# Autodesk Inventor assembly: Assembly8 (Cylinder Complete Sub Assembly)
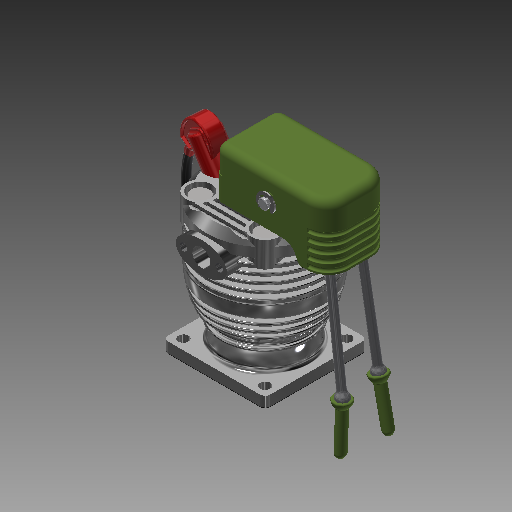
[picture p0: Inventor's stored thumbnail of the model, 512x512]
Saved by Autodesk Inventor 2018 (Build 220112000, 112)
## iProperties
Created: 2023-05-02
Part Number: Assembly8 (Cylinder Complete Sub Assembly)
Document SubType Name: Assembly
Designer: Habib Mohamed
Author: Habib Mohamed
## Documents named in this file (10)
- D:\Inventor\My projects\Rotary Engine\Assembly\Assembly8 (Cylinder Complete Sub Assembly).iam
- D:\Inventor\My projects\Rotary Engine\Component 48(Ignition Plug).ipt
- D:\Inventor\My projects\Rotary Engine\Component 45(Spark Plug).ipt
- D:\Inventor\My projects\Rotary Engine\Component 4 (Pound).ipt
- D:\Inventor\My projects\Rotary Engine\Component 39(Rod).ipt
- D:\Inventor\My projects\Rotary Engine\Assembly\Assembly7.iam
- Cykinder SubAssembly.iam
- D:\Inventor\My projects\Rotary Engine\Assembly\Assembly3(Rocker arm Sub Assembly).iam
- D:\Inventor\My projects\Rotary Engine\Assembly\Assembly5 (Valve Sub Assembly).iam
- D:\Inventor\My projects\Rotary Engine\Component 27 (Bracket Cover).ipt
## Components (12 placed, 8 different names)
1. Component 48(Ignition Plug):1 — Mate:1, Mate:2, Mate:3
2. Component 45(Spark Plug):1 — Mate:1, Mate:2, Mate:3, Mate:4, Mate:5
3. Component 4 (Pound):1 — Tangent:2
4. Component 39(Rod):1 — Tangent:2, Tangent:4
5. Component 4 (Pound):2 — Tangent:1
6. Component 39(Rod):2 — Tangent:1, Tangent:3
7. Cykinder SubAssembly:1 [sub-assembly] — Mate:4, Mate:5, Mate:6, Mate:7, Mate:8, Mate:9, Mate:10, Mate:11, Mate:12, Mate:13, Mate:14, Mate:15, Flush:1
8. Assembly3(Rocker arm Sub Assembly):1 [sub-assembly] — Mate:11, Mate:12, Tangent:4
9. Assembly5 (Valve Sub Assembly):1 [sub-assembly] — Mate:6, Mate:8
10. Assembly3(Rocker arm Sub Assembly):2 [sub-assembly] — Mate:10, Mate:13, Tangent:3
11. Assembly5 (Valve Sub Assembly):2 [sub-assembly] — Mate:7, Mate:9
12. Component 27 (Bracket Cover):1 — Mate:14, Mate:15, Flush:1
## Relationships (20: Mate 15, Tangent 4, Flush 1)
- Mate:1: Component 48(Ignition Plug):1 ↔ Component 45(Spark Plug):1
- Mate:2: Component 48(Ignition Plug):1 ↔ Component 45(Spark Plug):1
- Mate:3: Component 48(Ignition Plug):1 ↔ Component 45(Spark Plug):1
- Mate:4: Component 45(Spark Plug):1 ↔ Cykinder SubAssembly:1
- Mate:5: Component 45(Spark Plug):1 ↔ Cykinder SubAssembly:1
- Mate:6: Cykinder SubAssembly:1 ↔ Assembly5 (Valve Sub Assembly):1
- Mate:7: Cykinder SubAssembly:1 ↔ Assembly5 (Valve Sub Assembly):2
- Mate:8: Cykinder SubAssembly:1 ↔ Assembly5 (Valve Sub Assembly):1
- Mate:9: Cykinder SubAssembly:1 ↔ Assembly5 (Valve Sub Assembly):2
- Mate:10: Cykinder SubAssembly:1 ↔ Assembly3(Rocker arm Sub Assembly):2
- Mate:11: Cykinder SubAssembly:1 ↔ Assembly3(Rocker arm Sub Assembly):1
- Mate:12: Cykinder SubAssembly:1 ↔ Assembly3(Rocker arm Sub Assembly):1
- Mate:13: Cykinder SubAssembly:1 ↔ Assembly3(Rocker arm Sub Assembly):2
- Tangent:1: Component 4 (Pound):2 ↔ Component 39(Rod):2
- Tangent:2: Component 4 (Pound):1 ↔ Component 39(Rod):1
- Tangent:3: Component 39(Rod):2 ↔ Assembly3(Rocker arm Sub Assembly):2
- Tangent:4: Component 39(Rod):1 ↔ Assembly3(Rocker arm Sub Assembly):1
- Mate:14: Cykinder SubAssembly:1 ↔ Component 27 (Bracket Cover):1
- Mate:15: Cykinder SubAssembly:1 ↔ Component 27 (Bracket Cover):1
- Flush:1: Cykinder SubAssembly:1 ↔ Component 27 (Bracket Cover):1
